# Autodesk Inventor assembly: Assembled Water Sensor Chassi
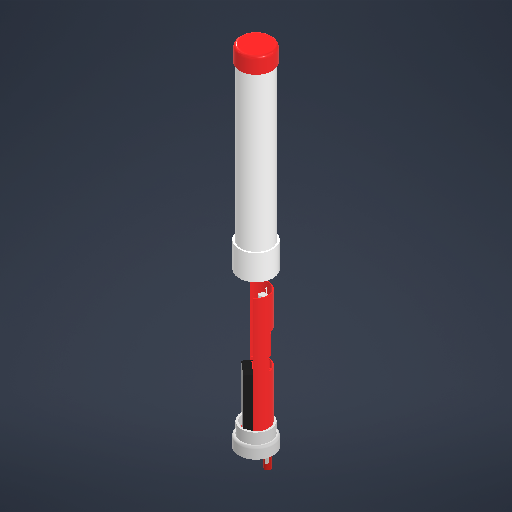
[picture p0: Inventor's stored thumbnail of the model, 512x512]
Saved by Autodesk Inventor 2026 (Build 300175050, 175E)
## iProperties
Created: 2024-06-24
Part Number: Assembled Water Sensor Chassi
Document SubType Name: Assembly
Designer: track
Author: track
## Documents named in this file (11)
- C:\Users\localuser\Documents\arts lab git\In-Situ-Water-Quality-Sensor\System_development\Jocassee\V0.5.1\Chassis\CAD model of Water Sensor\Assembled Water Sensor Chassi.iam
- C:\Users\localuser\Documents\arts lab git\In-Situ-Water-Quality-Sensor\System_development\Jocassee\V0.5.1\Chassis\CAD model of Water Sensor\Water_Sensor_Cap.ipt
- C:\Users\localuser\Documents\arts lab git\In-Situ-Water-Quality-Sensor\System_development\Jocassee\V0.5.1\Chassis\CAD model of Water Sensor\PCB tray CAD.ipt
- C:\Users\localuser\Documents\arts lab git\In-Situ-Water-Quality-Sensor\System_development\Jocassee\V0.4.7\Water Sensor Chassi CAD\Water Sensor Shaft (For assembly only).ipt
- C:\Users\localuser\Documents\arts lab git\In-Situ-Water-Quality-Sensor\System_development\Jocassee\V0.4.7\Water Sensor Chassi CAD\Male Adaptor to Water Sensor.ipt
- C:\Users\localuser\Documents\arts lab git\In-Situ-Water-Quality-Sensor\System_development\Jocassee\V0.4.7\Water Sensor Chassi CAD\Arc Water Sensor.ipt
- C:\Users\localuser\Documents\arts lab git\In-Situ-Water-Quality-Sensor\System_development\Jocassee\V0.4.7\Water Sensor Chassi CAD\Light Water Sensor.ipt
- C:\Users\localuser\Documents\arts lab git\In-Situ-Water-Quality-Sensor\System_development\Jocassee\V0.4.7\Water Sensor Chassi CAD\pH Sensor.ipt
- C:\Users\localuser\Documents\arts lab git\In-Situ-Water-Quality-Sensor\System_development\Jocassee\V0.4.7\Water Sensor Chassi CAD\Temp Water Sensor.ipt
- C:\Users\localuser\Documents\arts lab git\In-Situ-Water-Quality-Sensor\System_development\Jocassee\V0.4.7\Water Sensor Chassi CAD\Battery for Water Sensor.ipt
- C:\Users\localuser\Documents\arts lab git\In-Situ-Water-Quality-Sensor\System_development\Jocassee\V0.5.1\Chassis\CADs for Water Sensor assembly\PCB Board.ipt
## Components (10 placed, 10 different names)
1. PCB tray CAD:1 — Flush:2, Mate:2, Mate:6, Flush:5, Mate:11, Mate:12, Mate:16, Mate:17, Mate:18, Mate:19, Mate:20, Mate:21, Mate:22, Mate:23, Flush:6, Mate:24
2. Water Sensor Shaft (For assembly only):1 — Mate:14, Mate:15, Mate:25
3. Water_Sensor_Cap:1 — Mate:15, Mate:25
4. Male Adaptor to Water Sensor:1 — Mate:11, Mate:12, Mate:14
5. Arc Water Sensor:1 — Flush:5, Mate:16
6. Light Water Sensor:1 — Mate:20, Mate:21
7. pH Sensor:1 — Mate:6, Mate:17
8. Temp Water Sensor:1 — Flush:2, Mate:2
9. Battery for Water Sensor:1 — Mate:18, Mate:19, Mate:22
10. PCB Board:1 — Mate:23, Flush:6, Mate:24
## Relationships (19: Mate 16, Flush 3)
- Flush:2: PCB tray CAD:1 ↔ Temp Water Sensor:1
- Mate:2: PCB tray CAD:1 ↔ Temp Water Sensor:1
- Mate:6: PCB tray CAD:1 ↔ pH Sensor:1
- Flush:5: PCB tray CAD:1 ↔ Arc Water Sensor:1
- Mate:11: PCB tray CAD:1 ↔ Male Adaptor to Water Sensor:1
- Mate:12: PCB tray CAD:1 ↔ Male Adaptor to Water Sensor:1
- Mate:14: Water Sensor Shaft (For assembly only):1 ↔ Male Adaptor to Water Sensor:1
- Mate:15: Water Sensor Shaft (For assembly only):1 ↔ Water_Sensor_Cap:1
- Mate:16: PCB tray CAD:1 ↔ Arc Water Sensor:1
- Mate:17: PCB tray CAD:1 ↔ pH Sensor:1
- Mate:18: PCB tray CAD:1 ↔ Battery for Water Sensor:1
- Mate:19: PCB tray CAD:1 ↔ Battery for Water Sensor:1
- Mate:20: PCB tray CAD:1 ↔ Light Water Sensor:1
- Mate:21: PCB tray CAD:1 ↔ Light Water Sensor:1
- Mate:22 (5 mm): PCB tray CAD:1 ↔ Battery for Water Sensor:1
- Mate:23: PCB tray CAD:1 ↔ PCB Board:1
- Flush:6: PCB tray CAD:1 ↔ PCB Board:1
- Mate:24: PCB tray CAD:1 ↔ PCB Board:1
- Mate:25: Water Sensor Shaft (For assembly only):1 ↔ Water_Sensor_Cap:1
